# Autodesk Inventor assembly: foot-assembled
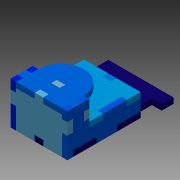
[picture p0: Inventor's stored thumbnail of the model, 180x180]
Saved by Autodesk Inventor 2013 (Build 170138000, 138)
## iProperties
Created: 2012-09-10
Part Number: foot-assembled
Document SubType Name: Assembly
Designer: frankenteddy
Author: frankenteddy
## Documents named in this file (8)
- C:\Users\frankenteddy\Desktop\oshawatt1\foot-assembled.iam
- C:\Users\frankenteddy\Desktop\oshawatt1\foot-back.ipt
- C:\Users\frankenteddy\Desktop\oshawatt1\foot-bottom.ipt
- C:\Users\frankenteddy\Desktop\oshawatt1\foot-front.ipt
- C:\Users\frankenteddy\Desktop\oshawatt1\foot-hip.ipt
- C:\Users\frankenteddy\Desktop\oshawatt1\foot-side.ipt
- C:\Users\frankenteddy\Desktop\oshawatt1\foot-toe.ipt
- C:\Users\frankenteddy\Desktop\oshawatt1\foot-top.ipt
## Components (8 placed, 7 different names)
1. foot-back:1 — Mate:1, Mate:2, Mate:3, Mate:9, Mate:17, Mate:24, Mate:25
2. foot-bottom:1 — Mate:9, Mate:11, Mate:12, Mate:13, Mate:22, Mate:23
3. foot-front:1 — Mate:4, Mate:6, Mate:18, Mate:19, Mate:20
4. foot-hip:1 — Mate:17, Mate:18, Mate:19
5. foot-side:1 — Mate:1, Mate:2, Mate:3, Mate:4, Mate:6, Mate:11, Mate:12, Mate:13, Mate:14, Mate:15, Mate:16, Mate:20, Mate:21
6. foot-toe:1 — Mate:21, Mate:22, Mate:23, Mate:26
7. foot-top:1 — Mate:14, Mate:15, Mate:16
8. foot-side:2 — Mate:24, Mate:25, Mate:26
## Relationships (22: Mate 22)
- Mate:1: foot-back:1 ↔ foot-side:1
- Mate:2: foot-back:1 ↔ foot-side:1
- Mate:3: foot-back:1 ↔ foot-side:1
- Mate:4: foot-front:1 ↔ foot-side:1
- Mate:6: foot-front:1 ↔ foot-side:1
- Mate:9: foot-back:1 ↔ foot-bottom:1
- Mate:11: foot-bottom:1 ↔ foot-side:1
- Mate:12: foot-bottom:1 ↔ foot-side:1
- Mate:13: foot-bottom:1 ↔ foot-side:1
- Mate:14: foot-side:1 ↔ foot-top:1
- Mate:15: foot-side:1 ↔ foot-top:1
- Mate:16: foot-side:1 ↔ foot-top:1
- Mate:17: foot-back:1 ↔ foot-hip:1
- Mate:18: foot-front:1 ↔ foot-hip:1
- Mate:19: foot-front:1 ↔ foot-hip:1
- Mate:20: foot-front:1 ↔ foot-side:1
- Mate:21: foot-side:1 ↔ foot-toe:1
- Mate:22: foot-bottom:1 ↔ foot-toe:1
- Mate:23: foot-bottom:1 ↔ foot-toe:1
- Mate:24: foot-back:1 ↔ foot-side:2
- Mate:25: foot-back:1 ↔ foot-side:2
- Mate:26: foot-toe:1 ↔ foot-side:2
